# Autodesk Inventor assembly: Assembly eyebrow
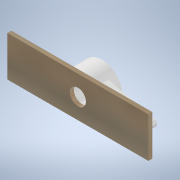
[picture p0: Inventor's stored thumbnail of the model, 180x180]
Saved by Autodesk Inventor 2021 (Build 250183000, 183)
## iProperties
Created: 2023-06-06
Part Number: Assembly eyebrow
Document SubType Name: Assembly
Designer: shrus
Author: shrus
## Documents named in this file (3)
- C:\Users\shrus\Documents\Assembly eyebrow.iam
- C:\Users\shrus\Documents\servoarm1.ipt
- C:\Users\shrus\Documents\Moving eyebrow.ipt
## Components (2 placed, 2 different names)
1. servoarm1:1 — Mate:1, Mate:2
2. Moving eyebrow:1 — Mate:1, Mate:2
## Relationships (2: Mate 2)
- Mate:1: servoarm1:1 ↔ Moving eyebrow:1
- Mate:2: servoarm1:1 ↔ Moving eyebrow:1
